# Autodesk Inventor assembly: Guntas_Belt_Wheel_Assembly
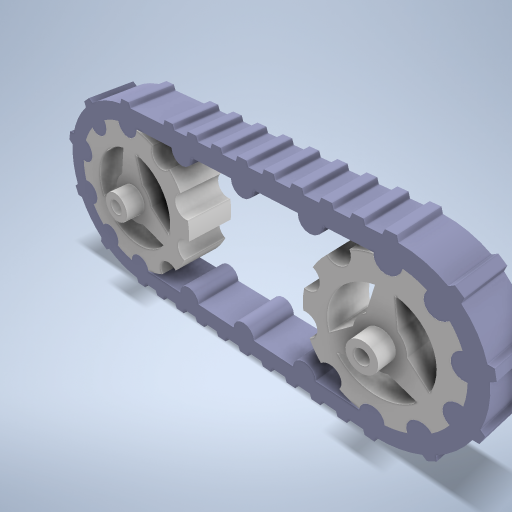
[picture p0: Inventor's stored thumbnail of the model, 512x512]
Saved by Autodesk Inventor 2024 (Build 280153000, 153)
## iProperties
Created: 2023-07-07
Part Number: Guntas_Belt_Wheel_Assembly
Document SubType Name: Assembly
Designer: manas
Author: manas
## Documents named in this file (3)
- D:\Parth Folder\ES101\Project\Wheels_Belt.iam
- D:\Parth Folder\ES101\Project\Belt.ipt
- D:\Parth Folder\ES101\Project\Wheel.ipt
## Components (3 placed, 2 different names)
1. Belt:1 — Mate:1, Flush:1, Mate:2, Flush:2
2. Wheel:1 — Mate:1, Flush:1
3. Wheel:2 — Mate:2, Flush:2
## Relationships (4: Mate 2, Flush 2)
- Mate:1: Belt:1 ↔ Wheel:1
- Flush:1: Belt:1 ↔ Wheel:1
- Mate:2: Belt:1 ↔ Wheel:2
- Flush:2: Belt:1 ↔ Wheel:2
